# Autodesk Inventor assembly: STHRANG10-MB
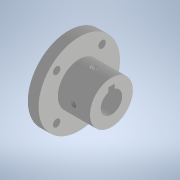
[picture p0: Inventor's stored thumbnail of the model, 180x180]
Saved by Autodesk Inventor 2021 (Build 250183000, 183)
## iProperties
Category: PARTsolutions
Company: MISUMI
Created: 2025-08-06
Part Number: STHRANG10-MB
Catalog Web Link: www.cadenas.de
Description: STHRBNG, STHRNG, SSTHRNG, STHRANG-Shaft Supports - with Damper - Key Groove - Round Flange
Vendor: MISUMI
Document SubType Name: Assembly
Designer: psAdmin
Manufacturer: MISUMI
Mass: 8.50205 g
Surface Area: 46.2101 cm^2
Volume: 8.50205 cm^3
Density: 1 g/cm^3
Title: STHRANG10-MB
Author: Cadenas PARTsolutions
Comments: Shaft Supports - with Damper - Key Groove - Round Flange
PSOL_IDENT_0: {$CADENAS_DATA/23d-libs/misumi/metric/02_shaft_supports/sthrbng_asmtab.prj},217 {VTYP=3D},{STYP=ASST
PSOL_IDENT_1: AB},{NB=STHRANG10-MB},{LINA=STHRANG10-MB},{NN=STHRBNG, STHRNG, SSTHRNG, STHRANG},{DATE=18.02.2024 14
PSOL_IDENT_2: :59:47},{GEOMDATE=16.02.2024 09:57:59},{VERSION=},{LINEID=210},{WBVAR=MAT,ST,ALT1},{WBNUMERIC=}  {NB=
PSOL_IDENT_3: STHRANG10-MB},{LINA=STHRANG10-MB},{KT=DUMMY},{PN=STHRANG10-MB},{TYPE=STHRANG},{MAT=5052},{MATALG= '1
PSOL_IDENT_4: 045', 'S45C Equivalent', '304', 'SUS304','5052','5052 Aluminum Alloy' },{ST=-},{D=10},{DTOL=+0.015/0
PSOL_IDENT_5: },{N=5.0},{L=20},{S=0},{L1=0},{D1=20},{H=38},{T=5},{LL=12},{M=M3},{THMD=3},{THDMIN=2.459},{P=30},{K=
PSOL_IDENT_6: 0},{W=20},{P1=30},{F=0},{DD1=4.5},{ST0='-','-'},{BB=3},{BBTOL=+0.013/-0.013},{TT=1.8},{TTTOL=+0.1/0}
PSOL_IDENT_7: ,{ALT1=MB},{MBM=M3},{ML=3},{ALT1PN=-MB},{PPATH=sthrbng/sthrbng_asmtpl.prj}
NB: STHRANG10-MB
NN: STHRBNG, STHRNG, SSTHRNG, STHRANG
NT: Shaft Supports - with Damper - Key Groove - Round Flange
NBSYN: $PN.
LINA: STHRANG10-MB
CATALOG: Misumi
PN: STHRANG10-MB
MAT: 5052 Aluminum Alloy
ST: -
D: 10
DTOL: +0.015/0
N: 5
L: 20
D1: 20
H: 38
T: 5
LL: 12
M: M3
P: 30
W: 20
P1: 30
F: 0
DD1: 4.5
BB: 3
BBTOL: +0.013/-0.013
TT: 1.8
TTTOL: +0.1/0
ALT1: with MB (Hex Socket Set Screw Included)
SUPPLIER: MISUMI
ARTICLENO: STHRANG10-MB
BOMINFO: STHRANG10-MB
CREATOR: CADENAS GmbH
## Documents named in this file (3)
- e:\temp\worker_COMMON_2\temp\tmp_3228_64_pwhLx\format_0\STHRANG10-MB.iam
- e:\temp\worker_COMMON_2\temp\tmp_3228_64_pwhLx\format_0\STHRANG10-MB_ss.ipt
- e:\temp\worker_COMMON_2\temp\tmp_3228_64_pwhLx\format_0\SET-SCREW3-3.ipt
## Components (3 placed, 2 different names)
1. STHRANG10-MB_ss:1 — to_screw1_XY@1 <-> CP_XY@2, to_screw1_Z@1 <-> CP_Z@2, to_screw1_YZ@1 <-> CP_YZ@2, to_screw2_XY@1 <-> CP_XY@3, to_screw2_Z@1 <-> CP_Z@3, to_screw2_YZ@1 <-> CP_YZ@3
2. SET-SCREW3-3:1 — to_screw1_XY@1 <-> CP_XY@2, to_screw1_Z@1 <-> CP_Z@2, to_screw1_YZ@1 <-> CP_YZ@2
3. SET-SCREW3-3:2 — to_screw2_XY@1 <-> CP_XY@3, to_screw2_Z@1 <-> CP_Z@3, to_screw2_YZ@1 <-> CP_YZ@3
## Relationships (6: Mate 4, Angle 2)
- to_screw1_XY@1 <-> CP_XY@2 [Mate]: STHRANG10-MB_ss:1 ↔ SET-SCREW3-3:1
- to_screw1_Z@1 <-> CP_Z@2 [Mate]: STHRANG10-MB_ss:1 ↔ SET-SCREW3-3:1
- to_screw1_YZ@1 <-> CP_YZ@2 [Angle] (0 deg): STHRANG10-MB_ss:1 ↔ SET-SCREW3-3:1
- to_screw2_XY@1 <-> CP_XY@3 [Mate]: STHRANG10-MB_ss:1 ↔ SET-SCREW3-3:2
- to_screw2_Z@1 <-> CP_Z@3 [Mate]: STHRANG10-MB_ss:1 ↔ SET-SCREW3-3:2
- to_screw2_YZ@1 <-> CP_YZ@3 [Angle] (0 deg): STHRANG10-MB_ss:1 ↔ SET-SCREW3-3:2
